# Autodesk Inventor assembly: Bumper_assey2
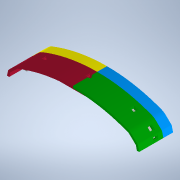
[picture p0: Inventor's stored thumbnail of the model, 180x180]
Saved by Autodesk Inventor 2020 (Build 240168000, 168)
## iProperties
Created: 2022-07-04
Part Number: Bumper_assey2
Document SubType Name: Assembly
Designer: SeungJin
Author: SeungJin
## Documents named in this file (7)
- C:\Users\SeungJin\Documents\Inventor\CoMoVi\Package\Bumper_assey2.iam
- C:\Users\SeungJin\Documents\Inventor\CoMoVi\Package\bumper_final_5.ipt
- C:\Users\SeungJin\Documents\Inventor\CoMoVi\Package\bumper_final_6.ipt
- C:\Users\SeungJin\Documents\Inventor\CoMoVi\Package\bumper_final_4.ipt
- C:\Users\SeungJin\Documents\Inventor\CoMoVi\Package\bumper_final_3.ipt
- C:\Users\SeungJin\Documents\Inventor\CoMoVi\Package\bumper_final_2.ipt
- C:\Users\SeungJin\Documents\Inventor\CoMoVi\Package\bumper_final_1.ipt
## Components (6 placed, 6 different names)
1. bumper_final_5:1 — 메이트:1, 플러쉬:1, 메이트:5, 메이트:6, 메이트:7
2. bumper_final_6:1 — 메이트:1, 플러쉬:1, 메이트:2, 메이트:3, 메이트:4
3. bumper_final_4:1 — 메이트:2, 메이트:3, 메이트:4, 메이트:12, 메이트:14
4. bumper_final_3:1 — 메이트:5, 메이트:6, 메이트:7, 메이트:11, 메이트:15
5. bumper_final_2:1 — 메이트:9, 메이트:10, 플러쉬:3, 메이트:12, 메이트:14
6. bumper_final_1:1 — 메이트:9, 메이트:10, 플러쉬:3, 메이트:11, 메이트:15
## Relationships (15: Mate 13, Flush 2)
- 메이트:1 [Mate]: bumper_final_5:1 ↔ bumper_final_6:1
- 플러쉬:1 [Flush]: bumper_final_5:1 ↔ bumper_final_6:1
- 메이트:2 [Mate]: bumper_final_6:1 ↔ bumper_final_4:1
- 메이트:3 [Mate]: bumper_final_6:1 ↔ bumper_final_4:1
- 메이트:4 [Mate]: bumper_final_6:1 ↔ bumper_final_4:1
- 메이트:5 [Mate]: bumper_final_5:1 ↔ bumper_final_3:1
- 메이트:6 [Mate]: bumper_final_5:1 ↔ bumper_final_3:1
- 메이트:7 [Mate]: bumper_final_5:1 ↔ bumper_final_3:1
- 메이트:9 [Mate]: bumper_final_2:1 ↔ bumper_final_1:1
- 메이트:10 [Mate]: bumper_final_2:1 ↔ bumper_final_1:1
- 플러쉬:3 [Flush]: bumper_final_2:1 ↔ bumper_final_1:1
- 메이트:11 [Mate]: bumper_final_3:1 ↔ bumper_final_1:1
- 메이트:12 [Mate]: bumper_final_4:1 ↔ bumper_final_2:1
- 메이트:14 [Mate]: bumper_final_4:1 ↔ bumper_final_2:1
- 메이트:15 [Mate]: bumper_final_3:1 ↔ bumper_final_1:1
